# Autodesk Inventor assembly: J005651
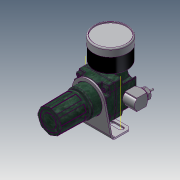
[picture p0: Inventor's stored thumbnail of the model, 180x180]
Saved by Autodesk Inventor 2015 SP1 (Build 190203100, 203)
## iProperties
Created: 2015-05-13
Vendor: HHMI: JRC - ID&F
Document SubType Name: Assembly
Designer: ARNOLDJ
Part Number: J005651
Description: REGULATOR AND GAUGE ASSY
RuleStatus: InUse
AfterDocSave0: file://Part Number Cleaner
DESIGN DEPARTMENT: HHMI: JRC - ID&F
ALTERED ITEM PART NUMBER: N/A
ALTERED ITEM VENDOR: N/A
ALTERED ITEM DESCRIPTION: N/A
Author: ARNOLDJ
Revision Number: 0
## Documents named in this file (7)
- C:\_WORKSPACE\DATA\COLLABORATION\SVOBODA LAB\MOUSE POSITIONING SYSTEMS\MCAD\BALL SETUP\MBS REGULATOR ASSY.iam
- C:\_WORKSPACE\DATA\COLLABORATION\SVOBODA LAB\MOUSE POSITIONING SYSTEMS\MCAD\BALL SETUP\MMR-2P.ipt
- C:\_WORKSPACE\DATA\COLLABORATION\SVOBODA LAB\MOUSE POSITIONING SYSTEMS\MCAD\BALL SETUP\MMH-B220.ipt
- C:\_WORKSPACE\DATA\COLLABORATION\SVOBODA LAB\MOUSE POSITIONING SYSTEMS\MCAD\BALL SETUP\5779K143.ipt
- C:\_WORKSPACE\DATA\COLLABORATION\SVOBODA LAB\MOUSE POSITIONING SYSTEMS\MCAD\BALL SETUP\PG-15-160P.ipt
- C:\_WORKSPACE\DATA\COLLABORATION\SVOBODA LAB\MOUSE POSITIONING SYSTEMS\MCAD\BALL SETUP\50785K410.ipt
- C:\_WORKSPACE\DATA\COLLABORATION\SVOBODA LAB\MOUSE POSITIONING SYSTEMS\MCAD\BALL SETUP\50745K150.ipt
## Components (6 placed, 6 different names)
1. MMR-2P:1 — Mate:1, Mate:2, Mate:3, Mate:4, Mate:5, Mate:6, Mate:7, Mate:8
2. MMH-B220:1 — Mate:1, Mate:2, Angle:1
3. 5779K143:1 — Mate:3, Mate:4
4. PG-15-160P:1 — Mate:5, Mate:6
5. 50785K410:1 — Mate:7, Mate:8, Mate:9, Mate:10
6. 50745K150:1 — Mate:9, Mate:10
## Relationships (11: Mate 10, Angle 1)
- Mate:1: MMR-2P:1 ↔ MMH-B220:1
- Mate:2: MMR-2P:1 ↔ MMH-B220:1
- Angle:1 (180 deg): MMH-B220:1
- Mate:3 (1.27 mm): MMR-2P:1 ↔ 5779K143:1
- Mate:4: MMR-2P:1 ↔ 5779K143:1
- Mate:5 (6.35 mm): MMR-2P:1 ↔ PG-15-160P:1
- Mate:6: MMR-2P:1 ↔ PG-15-160P:1
- Mate:7 (1.905 mm): MMR-2P:1 ↔ 50785K410:1
- Mate:8: MMR-2P:1 ↔ 50785K410:1
- Mate:9 (1.905 mm): 50785K410:1 ↔ 50745K150:1
- Mate:10: 50785K410:1 ↔ 50745K150:1
